# Autodesk Inventor assembly: Assembly4
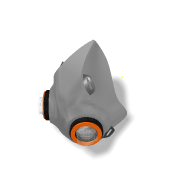
[picture p0: Inventor's stored thumbnail of the model, 180x180]
Saved by Autodesk Inventor 2021 (Build 250183000, 183)
## iProperties
Created: 2020-07-12
Part Number: Assembly4
Document SubType Name: Assembly
Designer: Derm
Author: Derm
## Documents named in this file (5)
- C:\Users\Derm\n95\v7\Assembly4.iam
- C:\Users\Derm\n95\v7\maskBodyV4Molds\thermoformedSupport.ipt
- C:\Users\Derm\n95\v7\3dpBayonetteMountV1Fastener.ipt
- C:\Users\Derm\n95\v7\3dpBayonetteMountV2.ipt
- C:\Users\Derm\n95\v7\outerMountGasket.ipt
## Components (7 placed, 4 different names)
1. thermoformedSupport:1 — Mate:3, Mate:6, Mate:7, Mate:8, Mate:11, Mate:12
2. 3dpBayonetteMountV1Fastener:1 — Mate:5, Mate:7, Mate:10
3. 3dpBayonetteMountV2:1 — Mate:4, Mate:5, Mate:6, Mate:11
4. outerMountGasket:1 — Mate:4, Mate:10
5. 3dpBayonetteMountV1Fastener:2 — Mate:2, Mate:8, Mate:9
6. 3dpBayonetteMountV2:2 — Mate:1, Mate:3, Mate:12
7. outerMountGasket:2 — Mate:1, Mate:2, Mate:9
## Relationships (12: Mate 12)
- Mate:1: 3dpBayonetteMountV2:2 ↔ outerMountGasket:2
- Mate:2: 3dpBayonetteMountV1Fastener:2 ↔ outerMountGasket:2
- Mate:3: thermoformedSupport:1 ↔ 3dpBayonetteMountV2:2
- Mate:4: 3dpBayonetteMountV2:1 ↔ outerMountGasket:1
- Mate:5: 3dpBayonetteMountV1Fastener:1 ↔ 3dpBayonetteMountV2:1
- Mate:6: thermoformedSupport:1 ↔ 3dpBayonetteMountV2:1
- Mate:7: thermoformedSupport:1 ↔ 3dpBayonetteMountV1Fastener:1
- Mate:8: thermoformedSupport:1 ↔ 3dpBayonetteMountV1Fastener:2
- Mate:9: 3dpBayonetteMountV1Fastener:2 ↔ outerMountGasket:2
- Mate:10: 3dpBayonetteMountV1Fastener:1 ↔ outerMountGasket:1
- Mate:11: thermoformedSupport:1 ↔ 3dpBayonetteMountV2:1
- Mate:12: thermoformedSupport:1 ↔ 3dpBayonetteMountV2:2
